# Autodesk Inventor assembly: Assembly1
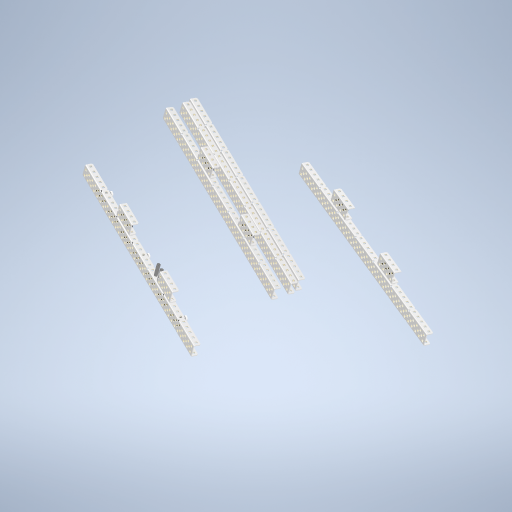
[picture p0: Inventor's stored thumbnail of the model, 512x512]
Saved by Autodesk Inventor 2023.2 (Build 272271000, 271)
## iProperties
Created: 2022-12-13
Part Number: Assembly1
Document SubType Name: Assembly
Designer: 76646426
Author: 76646426
## Documents named in this file (12)
- C:\Users\76646426\Downloads\Assembly1.iam
- C:\Users\Public\Documents\CAD\2021-2022 CAD Library\Structure\C-Channels\Aluminum 1x2x1\Alu C 1x2x1x35.ipt
- C:\Users\Public\Documents\CAD\2021-2022 CAD Library\Motion\Spacers\Spacer Nylon .313 OD\NSpacer .313 OD x .125.ipt
- C:\Users\Public\Documents\CAD\2021-2022 CAD Library\Motion\Spacers\Spacer Nylon .313 OD.ipt
- C:\Users\Public\Documents\CAD\2021-2022 CAD Library\Structure\C-Channels\Aluminum 1x2x1\Alu C 1x2x1x4.ipt
- C:\Users\Public\Documents\CAD\2021-2022 CAD Library\Motion\Bearing Flat.ipt
- C:\Users\76646426\Documents\9691A-Robot-Files\CAD\2021-2022 CAD Library\Structure\Standoff\Standoff 1.00.ipt
- C:\Users\76646426\Documents\9691A-Robot-Files\CAD\2021-2022 CAD Library\Structure\Standoff.ipt
- C:\Users\76646426\Documents\9691A-Robot-Files\CAD\2021-2022 CAD Library\Structure\Standoff\Standoff .50.ipt
- C:\Users\Public\Documents\CAD\2021-2022 CAD Library\Structure\C-Channels\Aluminum 1x2x1\Alu C 1x2x1x35_MIR.ipt
- C:\Users\Public\Documents\CAD\2021-2022 CAD Library\Structure\C-Channels\Aluminum 1x2x1\Alu C 1x2x1x4_MIR.ipt
- C:\Users\Public\Documents\CAD\2021-2022 CAD Library\Motion\Bearing Flat_MIR.ipt
## Components (42 placed, 9 different names)
1. Alu C 1x2x1x35:1 — Insert:6, Insert:8, Insert:10, Insert:12
2. NSpacer .313 OD x .125:1 — Insert:5, Insert:6
3. NSpacer .313 OD x .125:2 — Insert:7, Insert:8
4. Alu C 1x2x1x4:1 — Insert:3, Insert:4, Insert:5, Insert:7
5. NSpacer .313 OD x .125:3 — Insert:11, Insert:12
6. NSpacer .313 OD x .125:4 — Insert:9, Insert:10
7. Alu C 1x2x1x4:2 — Insert:1, Insert:2, Insert:9, Insert:11
8. Bearing Flat:1 — Insert:1, Insert:2
9. Bearing Flat:2 — Insert:3, Insert:4
10. Bearing Flat:3 — Insert:27, Insert:28
11. Bearing Flat:4 — Insert:21, Insert:22, Insert:23
12. Bearing Flat:5 — Insert:29, Insert:30, Insert:32
13. Bearing Flat:6 — Insert:25, Insert:26
14. Alu C 1x2x1x35:2 — Insert:13, Insert:14, Insert:17, Insert:18, Insert:19, Insert:20, Insert:21, Insert:22, Insert:25, Insert:26, Insert:27, Insert:28, Insert:29, Insert:30
15. NSpacer .313 OD x .125:5
16. NSpacer .313 OD x .125:6
17. Alu C 1x2x1x4:3
18. NSpacer .313 OD x .125:7
19. Alu C 1x2x1x4:4
20. Bearing Flat:7
21. Standoff 1.00:1
22. Standoff 1.00:2
23. Standoff .50:3 — Insert:15, Insert:16
24. Standoff .50:4 — Insert:23, Insert:24
25. Standoff .50:5 — Insert:31, Insert:32
26. NSpacer .313 OD x .125:8 — Insert:31
27. NSpacer .313 OD x .125:9 — Insert:24
28. NSpacer .313 OD x .125:10 — Insert:16
29. Bearing Flat:8 — Insert:13, Insert:14, Insert:15
30. Bearing Flat:9 — Insert:17, Insert:19
31. Bearing Flat:10 — Insert:18, Insert:20
32. Alu C 1x2x1x35:3
33. Alu C 1x2x1x35:4
34. Alu C 1x2x1x35_MIR:1 — Insert:33, Insert:34, Insert:37, Insert:38
35. NSpacer .313 OD x .125:11 — Insert:33, Insert:36
36. NSpacer .313 OD x .125:12 — Insert:34, Insert:35
37. Alu C 1x2x1x4_MIR:1 — Insert:35, Insert:36, Insert:43, Insert:44
38. NSpacer .313 OD x .125:13 — Insert:37, Insert:39
39. NSpacer .313 OD x .125:14 — Insert:38, Insert:40
40. Alu C 1x2x1x4_MIR:2 — Insert:39, Insert:40, Insert:41, Insert:42
41. Bearing Flat_MIR:1 — Insert:41, Insert:42
42. Bearing Flat_MIR:2 — Insert:43, Insert:44
## Relationships (65: Insert 44, Mate 21)
- Insert:1: Alu C 1x2x1x4:2 ↔ Bearing Flat:1
- Insert:2: Alu C 1x2x1x4:2 ↔ Bearing Flat:1
- Insert:3: Alu C 1x2x1x4:1 ↔ Bearing Flat:2
- Insert:4: Alu C 1x2x1x4:1 ↔ Bearing Flat:2
- Insert:5: NSpacer .313 OD x .125:1 ↔ Alu C 1x2x1x4:1
- Insert:6: Alu C 1x2x1x35:1 ↔ NSpacer .313 OD x .125:1
- Insert:7: NSpacer .313 OD x .125:2 ↔ Alu C 1x2x1x4:1
- Insert:8: Alu C 1x2x1x35:1 ↔ NSpacer .313 OD x .125:2
- Insert:9: NSpacer .313 OD x .125:4 ↔ Alu C 1x2x1x4:2
- Insert:10: Alu C 1x2x1x35:1 ↔ NSpacer .313 OD x .125:4
- Insert:11: NSpacer .313 OD x .125:3 ↔ Alu C 1x2x1x4:2
- Insert:12: Alu C 1x2x1x35:1 ↔ NSpacer .313 OD x .125:3
- [Mate]: Alu C 1x2x1x35:2 ↔ NSpacer .313 OD x .125:6
- [Mate]: Alu C 1x2x1x35:2 ↔ NSpacer .313 OD x .125:5
- [Mate]: Alu C 1x2x1x35:2 ↔ NSpacer .313 OD x .125:6
- [Mate]: Alu C 1x2x1x35:2 ↔ NSpacer .313 OD x .125:5
- [Mate]: NSpacer .313 OD x .125:5 ↔ Alu C 1x2x1x4:3
- [Mate]: NSpacer .313 OD x .125:6 ↔ Alu C 1x2x1x4:3
- [Mate]: NSpacer .313 OD x .125:6 ↔ Alu C 1x2x1x4:3
- [Mate]: Alu C 1x2x1x35:2 ↔ NSpacer .313 OD x .125:7
- [Mate]: Alu C 1x2x1x35:2 ↔ NSpacer .313 OD x .125:7
- [Mate]: NSpacer .313 OD x .125:7 ↔ Alu C 1x2x1x4:4
- [Mate]: NSpacer .313 OD x .125:7 ↔ Alu C 1x2x1x4:4
- [Mate]: NSpacer .313 OD x .125:7 ↔ Alu C 1x2x1x4:4
- [Mate]: Alu C 1x2x1x4:3 ↔ Bearing Flat:7
- [Mate]: Alu C 1x2x1x4:3 ↔ Bearing Flat:7
- [Mate]: Alu C 1x2x1x4:3 ↔ Bearing Flat:7
- [Mate]: Alu C 1x2x1x35:2 ↔ Standoff 1.00:2
- [Mate]: Alu C 1x2x1x35:2 ↔ Standoff 1.00:1
- [Mate]: Alu C 1x2x1x35:2 ↔ Standoff 1.00:1
- [Mate]: Alu C 1x2x1x35:2 ↔ Standoff 1.00:2
- [Mate]: Standoff .50:5 ↔ NSpacer .313 OD x .125:8
- [Mate]: Standoff .50:5 ↔ NSpacer .313 OD x .125:8
- Insert:13: Alu C 1x2x1x35:2 ↔ Bearing Flat:8
- Insert:14: Alu C 1x2x1x35:2 ↔ Bearing Flat:8
- Insert:15: Standoff .50:3 ↔ Bearing Flat:8
- Insert:16: Standoff .50:3 ↔ NSpacer .313 OD x .125:10
- Insert:17: Alu C 1x2x1x35:2 ↔ Bearing Flat:9
- Insert:18: Alu C 1x2x1x35:2 ↔ Bearing Flat:10
- Insert:19: Alu C 1x2x1x35:2 ↔ Bearing Flat:9
- Insert:20: Alu C 1x2x1x35:2 ↔ Bearing Flat:10
- Insert:21: Bearing Flat:4 ↔ Alu C 1x2x1x35:2
- Insert:22: Bearing Flat:4 ↔ Alu C 1x2x1x35:2
- Insert:23: Bearing Flat:4 ↔ Standoff .50:4
- Insert:24: Standoff .50:4 ↔ NSpacer .313 OD x .125:9
- Insert:25: Bearing Flat:6 ↔ Alu C 1x2x1x35:2
- Insert:26: Bearing Flat:6 ↔ Alu C 1x2x1x35:2
- Insert:27: Bearing Flat:3 ↔ Alu C 1x2x1x35:2
- Insert:28: Bearing Flat:3 ↔ Alu C 1x2x1x35:2
- Insert:29: Bearing Flat:5 ↔ Alu C 1x2x1x35:2
- Insert:30: Bearing Flat:5 ↔ Alu C 1x2x1x35:2
- Insert:31: Standoff .50:5 ↔ NSpacer .313 OD x .125:8
- Insert:32: Bearing Flat:5 ↔ Standoff .50:5
- Insert:33: Alu C 1x2x1x35_MIR:1 ↔ NSpacer .313 OD x .125:11
- Insert:34: Alu C 1x2x1x35_MIR:1 ↔ NSpacer .313 OD x .125:12
- Insert:35: NSpacer .313 OD x .125:12 ↔ Alu C 1x2x1x4_MIR:1
- Insert:36: NSpacer .313 OD x .125:11 ↔ Alu C 1x2x1x4_MIR:1
- Insert:37: Alu C 1x2x1x35_MIR:1 ↔ NSpacer .313 OD x .125:13
- Insert:38: Alu C 1x2x1x35_MIR:1 ↔ NSpacer .313 OD x .125:14
- Insert:39: NSpacer .313 OD x .125:13 ↔ Alu C 1x2x1x4_MIR:2
- Insert:40: NSpacer .313 OD x .125:14 ↔ Alu C 1x2x1x4_MIR:2
- Insert:41: Alu C 1x2x1x4_MIR:2 ↔ Bearing Flat_MIR:1
- Insert:42: Alu C 1x2x1x4_MIR:2 ↔ Bearing Flat_MIR:1
- Insert:43: Alu C 1x2x1x4_MIR:1 ↔ Bearing Flat_MIR:2
- Insert:44: Alu C 1x2x1x4_MIR:1 ↔ Bearing Flat_MIR:2
